# Autodesk Inventor assembly: Third Arm
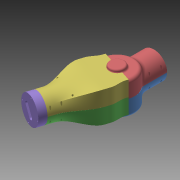
[picture p0: Inventor's stored thumbnail of the model, 180x180]
Saved by Autodesk Inventor 2015 (Build 190159000, 159)
## iProperties
Created: 2015-12-04
Part Number: Third Arm
Document SubType Name: Assembly
Designer: Eli
Author: Eli
## Documents named in this file (6)
- C:\Users\Eli\Desktop\School\15-16 Fall\VIP RM\Third Arm.iam
- C:\Users\Eli\Desktop\School\15-16 Fall\VIP RM\Upper Arm Top.ipt
- C:\Users\Eli\Desktop\School\15-16 Fall\VIP RM\Upper Arm Bottom.ipt
- C:\Users\Eli\Desktop\School\15-16 Fall\VIP RM\Lower Arm Top.ipt
- C:\Users\Eli\Desktop\School\15-16 Fall\VIP RM\Lower Arm Bottom1.ipt
- C:\Users\Eli\Desktop\School\15-16 Fall\VIP RM\Arm Plate.ipt
## Components (5 placed, 5 different names)
1. Upper Arm Top:1 — Mate:1, Flush:1, Flush:2, Mate:3, Mate:4, Mate:7, Mate:8
2. Upper Arm Bottom:1 — Mate:1, Flush:1, Flush:2
3. Lower Arm Top:1 — Mate:3, Mate:4, Mate:5, Mate:6, Flush:3, Mate:7, Mate:8, Mate:9, Mate:10
4. Lower Arm Bottom1:1 — Mate:5, Mate:6, Flush:3
5. Arm Plate:1 — Mate:9, Mate:10
## Relationships (12: Mate 9, Flush 3)
- Mate:1: Upper Arm Top:1 ↔ Upper Arm Bottom:1
- Flush:1: Upper Arm Top:1 ↔ Upper Arm Bottom:1
- Flush:2: Upper Arm Top:1 ↔ Upper Arm Bottom:1
- Mate:3: Upper Arm Top:1 ↔ Lower Arm Top:1
- Mate:4: Upper Arm Top:1 ↔ Lower Arm Top:1
- Mate:5: Lower Arm Top:1 ↔ Lower Arm Bottom1:1
- Mate:6: Lower Arm Top:1 ↔ Lower Arm Bottom1:1
- Flush:3: Lower Arm Top:1 ↔ Lower Arm Bottom1:1
- Mate:7: Upper Arm Top:1 ↔ Lower Arm Top:1
- Mate:8: Upper Arm Top:1 ↔ Lower Arm Top:1
- Mate:9: Lower Arm Top:1 ↔ Arm Plate:1
- Mate:10: Lower Arm Top:1 ↔ Arm Plate:1
